# Autodesk Inventor assembly: gearTry01
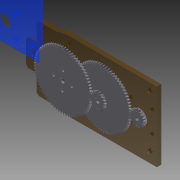
[picture p0: Inventor's stored thumbnail of the model, 180x180]
Saved by Autodesk Inventor 2013 (Build 170138000, 138)
## iProperties
Created: 2014-07-01
Part Number: gearTry01
Document SubType Name: Assembly
Designer: Nano
Author: Nano
## Documents named in this file (4)
- C:\Users\Nano\Documents\InventorByron\InventorMasterProject\panTiltSystem\gearExperiments\gearTry01.iam
- C:\Users\Nano\Documents\InventorByron\InventorMasterProject\panTiltSystem\gearExperiments\gearTry01\Design Accelerator\Spur Gears1.iam
- C:\Users\Nano\Documents\InventorByron\InventorMasterProject\panTiltSystem\gearExperiments\gearTry01\Design Accelerator\Spur Gears21.iam
- C:\Users\Nano\Documents\InventorByron\InventorMasterProject\panTiltSystem\gearExperiments\gearBoxBaseTilt.ipt
## Components (3 placed, 3 different names)
1. gearBoxBaseTilt:1 — Mate:3, Mate:7, Mate:8, Mate:9, Mate:10
2. Spur Gears:1 [sub-assembly] — Mate:3, Mate:6, Rotation:1, Mate:7, Mate:8
3. Spur Gears2:2 [sub-assembly] — Mate:6, Rotation:1, Mate:9, Mate:10
## Relationships (7: Mate 6, RelateRotation 1)
- Mate:3 (1.016 mm): gearBoxBaseTilt:1 ↔ Spur Gears:1
- Mate:6 (3.175 mm): Spur Gears:1 ↔ Spur Gears2:2
- Rotation:1 [RelateRotation] (1 ul): Spur Gears:1 ↔ Spur Gears2:2
- Mate:7: gearBoxBaseTilt:1 ↔ Spur Gears:1
- Mate:8: gearBoxBaseTilt:1 ↔ Spur Gears:1
- Mate:9: gearBoxBaseTilt:1 ↔ Spur Gears2:2
- Mate:10: gearBoxBaseTilt:1 ↔ Spur Gears2:2
